# Autodesk Inventor assembly: GINBAL2.2
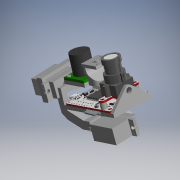
[picture p0: Inventor's stored thumbnail of the model, 180x180]
Saved by Autodesk Inventor 2019 (Build 230136000, 136)
## iProperties
Created: 2020-03-28
Part Number: GINBAL2.2
Document SubType Name: Assembly
Designer: Pulag
Author: Pulag
## Documents named in this file (7)
- C:\Users\Pulag\Documents\GitHub\24th_TDK_Project_D5\CAD\frame\GIMBAL\GINBAL2.2.iam
- C:\Users\Pulag\Documents\GitHub\24th_TDK_Project_D5\CAD\Syno_borad_3D\匯出\SG90.ipt
- C:\Users\Pulag\Documents\GitHub\24th_TDK_Project_D5\CAD\frame\LPATFORM.ipt
- C:\Users\Pulag\Documents\GitHub\24th_TDK_Project_D5\CAD\CAD file\OpenMV H7\openmv4_h7.iam
- C:\Users\Pulag\Documents\GitHub\24th_TDK_Project_D5\CAD\frame\SONIC.ipt
- C:\Users\Pulag\Documents\GitHub\24th_TDK_Project_D5\CAD\frame\optical.ipt
- C:\Users\Pulag\Documents\GitHub\24th_TDK_Project_D5\CAD\frame\armv3.ipt
## Components (7 placed, 6 different names)
1. SG90:1 — Mate:19, Mate:20
2. SG90:2 — Mate:14, Flush:13, Mate:21, Mate:22, Mate:23
3. LPATFORM:1 — Flush:4, Mate:13, Mate:14, Mate:16, Flush:13
4. openmv4_h7:1 [sub-assembly] — Angle:4, Flush:2, Flush:3, Flush:4, Mate:13, Mate:16, Mate:17
5. SONIC:1 — Angle:4, Flush:2, Flush:3, Angle:5, Flush:8, Flush:9, Mate:18
6. optical:1 — Angle:5, Flush:8, Flush:9, Mate:17, Mate:18
7. armv3:1 — Mate:19, Mate:20, Mate:21, Mate:22, Mate:23
## Relationships (18: Mate 10, Flush 6, Angle 2)
- Angle:4 (180 deg): openmv4_h7:1 ↔ SONIC:1
- Flush:2: openmv4_h7:1 ↔ SONIC:1
- Flush:3 (6.78 mm): openmv4_h7:1 ↔ SONIC:1
- Flush:4: LPATFORM:1 ↔ openmv4_h7:1
- Mate:13: LPATFORM:1 ↔ openmv4_h7:1
- Mate:14: SG90:2 ↔ LPATFORM:1
- Mate:16: LPATFORM:1 ↔ openmv4_h7:1
- Angle:5 (0 deg): SONIC:1 ↔ optical:1
- Flush:8 (4 mm): SONIC:1 ↔ optical:1
- Flush:9 (10 mm): SONIC:1 ↔ optical:1
- Mate:17 (0.674 mm): openmv4_h7:1 ↔ optical:1
- Mate:18 (0.132 mm): SONIC:1 ↔ optical:1
- Flush:13: SG90:2 ↔ LPATFORM:1
- Mate:19: SG90:1 ↔ armv3:1
- Mate:20: SG90:1 ↔ armv3:1
- Mate:21: SG90:2 ↔ armv3:1
- Mate:22: SG90:2 ↔ armv3:1
- Mate:23: SG90:2 ↔ armv3:1
